# Autodesk Inventor assembly: 回転アームテスト
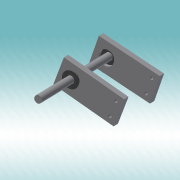
[picture p0: Inventor's stored thumbnail of the model, 180x180]
Saved by Autodesk Inventor 2015 (Build 190159000, 159)
## iProperties
Created: 2016-03-21
Part Number: 回転アームテスト
Document SubType Name: 溶接アセンブリ
Designer: buzztaka
Weld Material: アルミニウム 6061、溶接
Author: buzztaka
## Documents named in this file (4)
- C:\Users\buzztaka\Documents\tukuba\i-cart-middle_3d-model\計測輪アセンブル\回転アームテスト.iam
- C:\Users\buzztaka\Documents\tukuba\i-cart-middle_3d-model\計測輪アセンブル\回転軸取り付け板.ipt
- C:\Users\buzztaka\Documents\tukuba\i-cart-middle_3d-model\計測輪アセンブル\C-SFL6901ZZ.ipt
- C:\Users\buzztaka\Documents\tukuba\i-cart-middle_3d-model\計測輪アセンブル\回転軸.ipt
## Components (5 placed, 3 different names)
1. 回転軸取り付け板:1 — 挿入:1
2. C-SFL6901ZZ:1 — 挿入:1, 挿入:4
3. 回転軸取り付け板:2
4. C-SFL6901ZZ:2 — 挿入:3
5. 回転軸:1 — 挿入:3, 挿入:4
## Relationships (4: Insert 4)
- 挿入:1 [Insert]: 回転軸取り付け板:1 ↔ C-SFL6901ZZ:1
- [Insert]: 回転軸取り付け板:2 ↔ C-SFL6901ZZ:2
- 挿入:3 [Insert] (10 mm): C-SFL6901ZZ:2 ↔ 回転軸:1
- 挿入:4 [Insert] (-105 mm): C-SFL6901ZZ:1 ↔ 回転軸:1
## Named parameters: d1_d0 = 0 mm
